# Autodesk Inventor assembly: dc Motor
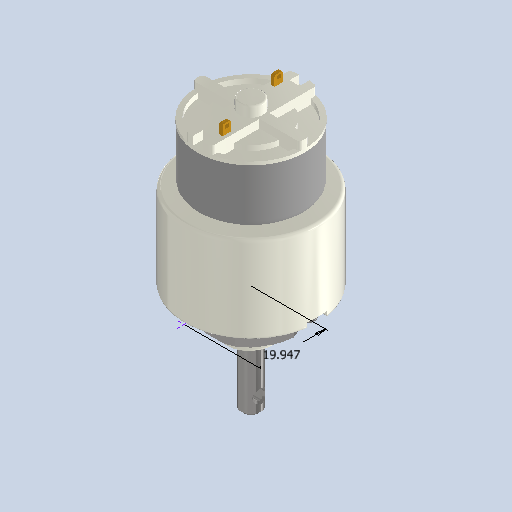
[picture p0: Inventor's stored thumbnail of the model, 512x512]
Saved by Autodesk Inventor 2024 (Build 280153000, 153)
## iProperties
Created: 2021-08-06
Part Number: dc Motor
Document SubType Name: Assembly
Designer: Suriyan.S
Author: Suriyan.S
## Documents named in this file (3)
- C:\Users\shraa\Downloads\Useless machine assembly\dc Motor.iam
- C:\Users\shraa\Downloads\Useless machine assembly\Nut (2).ipt
- C:\Users\shraa\Downloads\Useless machine assembly\Wheel Gear Motor.ipt
## Components (2 placed, 2 different names)
1. Nut (2):1 — Mate:1, Mate:2
2. Wheel Gear Motor:1 — Mate:1, Mate:2
## Relationships (2: Mate 2)
- Mate:1: Nut (2):1 ↔ Wheel Gear Motor:1
- Mate:2: Nut (2):1 ↔ Wheel Gear Motor:1
